# Autodesk Inventor assembly: Assembly fork ver2
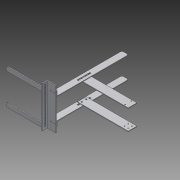
[picture p0: Inventor's stored thumbnail of the model, 180x180]
Saved by Autodesk Inventor 2015 (Build 190159000, 159)
## iProperties
Created: 2015-06-22
Part Number: Assembly fork ver2
Document SubType Name: Assembly
Designer: kenta
Mass: 58.3199 g
Surface Area: 327.704 cm^2
Volume: 21.7612 cm^3
Density: 2.68 g/cm^3
Author: kenta
## Documents named in this file (7)
- C:\Users\kenta\Documents\Inventor\知能ロボコン\Fork ver2\Assembly fork ver2.iam
- C:\Users\kenta\Documents\Inventor\知能ロボコン\Fork ver2\Fork 3 ver2.ipt
- C:\Users\kenta\Documents\Inventor\知能ロボコン\Fork ver2\Fork 1 left ver2.ipt
- C:\Users\kenta\Documents\Inventor\知能ロボコン\Fork ver2\Fork 1 right ver2.ipt
- C:\Users\kenta\Documents\Inventor\知能ロボコン\Fork ver2\Fork 2 ver2.ipt
- C:\Users\kenta\Documents\Inventor\知能ロボコン\Fork ver2\Fork 4 left ver2.ipt
- C:\Users\kenta\Documents\Inventor\知能ロボコン\Fork ver2\Fork 4 right ver2.ipt
## Components (7 placed, 6 different names)
1. Fork 3 ver2:1 — 挿入:1, 挿入:2
2. Fork 3 ver2:2 — 挿入:3, 挿入:4, メイト:3
3. Fork 1 left ver2:1 — メイト:1, フラッシュ:7
4. Fork 1 right ver2:1 — メイト:2, フラッシュ:8
5. Fork 2 ver2:1 — 挿入:1, 挿入:2, 挿入:3, 挿入:4, メイト:1, メイト:2, フラッシュ:7, フラッシュ:8
6. Fork 4 left ver2:1 — 挿入:5, 挿入:6
7. Fork 4 right ver2:1 — 挿入:5, 挿入:6, メイト:3
## Relationships (11: Insert 6, Mate 3, Flush 2)
- 挿入:1 [Insert]: Fork 3 ver2:1 ↔ Fork 2 ver2:1
- 挿入:2 [Insert]: Fork 3 ver2:1 ↔ Fork 2 ver2:1
- 挿入:3 [Insert]: Fork 3 ver2:2 ↔ Fork 2 ver2:1
- 挿入:4 [Insert]: Fork 3 ver2:2 ↔ Fork 2 ver2:1
- メイト:1 [Mate]: Fork 1 left ver2:1 ↔ Fork 2 ver2:1
- メイト:2 [Mate]: Fork 1 right ver2:1 ↔ Fork 2 ver2:1
- 挿入:5 [Insert] (45 mm): Fork 4 left ver2:1 ↔ Fork 4 right ver2:1
- 挿入:6 [Insert] (45 mm): Fork 4 left ver2:1 ↔ Fork 4 right ver2:1
- メイト:3 [Mate]: Fork 3 ver2:2 ↔ Fork 4 right ver2:1
- フラッシュ:7 [Flush]: Fork 1 left ver2:1 ↔ Fork 2 ver2:1
- フラッシュ:8 [Flush]: Fork 1 right ver2:1 ↔ Fork 2 ver2:1
